# Autodesk Inventor assembly: Assembly1
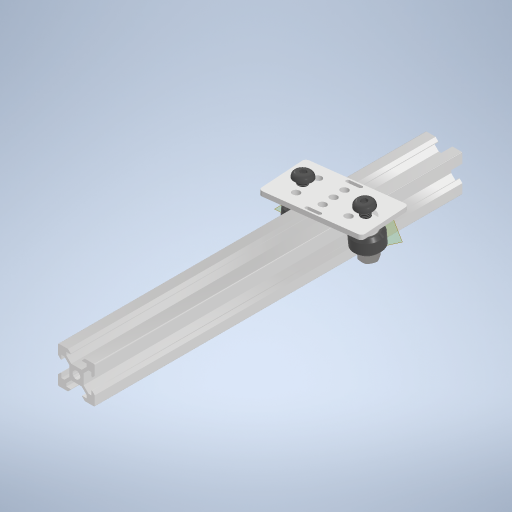
[picture p0: Inventor's stored thumbnail of the model, 512x512]
Saved by Autodesk Inventor 2024 (Build 280153000, 153)
## iProperties
Created: 2024-12-08
Part Number: Assembly1
Document SubType Name: Assembly
Designer: Nada
Author: Nada
## Documents named in this file (4)
- C:\Users\Adham\Documents\Modeling model\Modeling model\Assembly1.iam
- C:\Users\Adham\Documents\Modeling model\Modeling model\Cart.ipt
- C:\Users\Adham\Documents\Modeling model\Modeling model\Perfil2020.ipt
- C:\Users\Adham\Documents\Modeling model\Modeling model\Delrin Mini V-Wheel.iam
## Components (4 placed, 3 different names)
1. Cart:1 — Insert:1
2. Perfil2020:1 — Mate:1, Mate:2
3. Delrin Mini V-Wheel:1 [sub-assembly] — Mate:2
4. Delrin Mini V-Wheel:2 [sub-assembly] — Mate:1, Insert:1
## Relationships (3: Mate 2, Insert 1)
- Mate:1 (6 mm): Perfil2020:1 ↔ Delrin Mini V-Wheel:2
- Insert:1: Cart:1 ↔ Delrin Mini V-Wheel:2
- Mate:2 (6 mm): Perfil2020:1 ↔ Delrin Mini V-Wheel:1
